# Autodesk Inventor assembly: Motor_suj
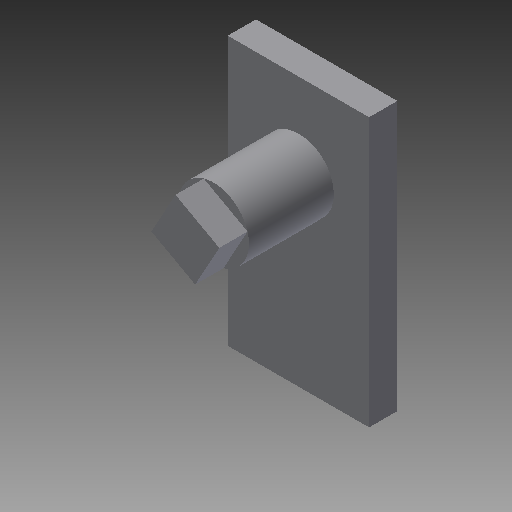
[picture p0: Inventor's stored thumbnail of the model, 512x512]
Saved by Autodesk Inventor 2018 (Build 220112000, 112)
## iProperties
Created: 2021-07-09
Part Number: Motor_suj
Material: Genérico
Document SubType Name: Assembly
Designer: GABRIEL
Author: GABRIEL
## Documents named in this file (3)
- C:\Users\GABRIEL\Documents\Gabriel\UNAL\SEMESTRE XI\Automatización de PM\Proyecto\Maquina de boca de pescado\Motor_suj.iam
- C:\Users\GABRIEL\Documents\Gabriel\UNAL\SEMESTRE XI\Automatización de PM\Proyecto\Maquina de boca de pescado\BaseM.ipt
- C:\Users\GABRIEL\Documents\Gabriel\UNAL\SEMESTRE XI\Automatización de PM\Proyecto\Maquina de boca de pescado\ejeM.ipt
## Components (2 placed, 2 different names)
1. BaseM:1 — Coincidencia:1, Nivelación:1
2. ejeM:1 — Coincidencia:1, Nivelación:1
## Relationships (2: Mate 1, Flush 1)
- Coincidencia:1 [Mate]: BaseM:1 ↔ ejeM:1
- Nivelación:1 [Flush]: BaseM:1 ↔ ejeM:1
